# Autodesk Inventor assembly: pulley 48 tooth + hub
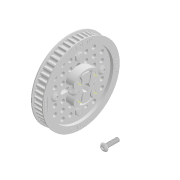
[picture p0: Inventor's stored thumbnail of the model, 180x180]
Saved by Autodesk Inventor 2020 (Build 240168000, 168)
## iProperties
Created: 2020-02-22
Part Number: pulley 48 tooth + hub
Document SubType Name: Assembly
Designer: ball
Author: ball
## Documents named in this file (5)
- C:\FTC\FTC8863CAD\2019 Robot\Mecanum Drive Train Metal\pulley 48 tooth + hub.iam
- C:\FTC\FTC8863CAD\GoBilda\3415 Parts\3415-0014-0048 Assembly.ipt
- C:\FTC\FTC8863CAD\GoBilda\1309 Parts\1309-0016-4008 assembly.ipt
- C:\FTC\FTC8863CAD\StepLibraries\Screws\M4 x 14 SOCKET HEAD CAP SCREW.ipt
- C:\FTC\FTC8863CAD\StepLibraries\Screws\M4 x 14 BUTTON HEAD HEX DRIVE SCREW.ipt
## Components (7 placed, 4 different names)
1. 3415-0014-0048 Assembly:1 — Mate:1, Mate:2, Flush:1, Mate:3, Mate:5, Mate:7, Mate:9
2. 1309-0016-4008 assembly:1 — Mate:1, Mate:2, Flush:1, Mate:4, Mate:6, Mate:8, Mate:10
3. M4 x 14 SOCKET HEAD CAP SCREW:1 — Mate:3, Mate:4
4. M4 x 14 SOCKET HEAD CAP SCREW:2 — Mate:7, Mate:8
5. M4 x 14 SOCKET HEAD CAP SCREW:3 — Mate:5, Mate:6
6. M4 x 14 SOCKET HEAD CAP SCREW:4 — Mate:9, Mate:10
7. M4 x 14 BUTTON HEAD HEX DRIVE SCREW:1
## Relationships (11: Mate 10, Flush 1)
- Mate:1: 3415-0014-0048 Assembly:1 ↔ 1309-0016-4008 assembly:1
- Mate:2: 3415-0014-0048 Assembly:1 ↔ 1309-0016-4008 assembly:1
- Flush:1: 3415-0014-0048 Assembly:1 ↔ 1309-0016-4008 assembly:1
- Mate:3: 3415-0014-0048 Assembly:1 ↔ M4 x 14 SOCKET HEAD CAP SCREW:1
- Mate:4: 1309-0016-4008 assembly:1 ↔ M4 x 14 SOCKET HEAD CAP SCREW:1
- Mate:5: 3415-0014-0048 Assembly:1 ↔ M4 x 14 SOCKET HEAD CAP SCREW:3
- Mate:6: 1309-0016-4008 assembly:1 ↔ M4 x 14 SOCKET HEAD CAP SCREW:3
- Mate:7: 3415-0014-0048 Assembly:1 ↔ M4 x 14 SOCKET HEAD CAP SCREW:2
- Mate:8: 1309-0016-4008 assembly:1 ↔ M4 x 14 SOCKET HEAD CAP SCREW:2
- Mate:9: 3415-0014-0048 Assembly:1 ↔ M4 x 14 SOCKET HEAD CAP SCREW:4
- Mate:10: 1309-0016-4008 assembly:1 ↔ M4 x 14 SOCKET HEAD CAP SCREW:4
